# Autodesk Inventor assembly: 3 in 30A flex wheel 36t gear HS mount
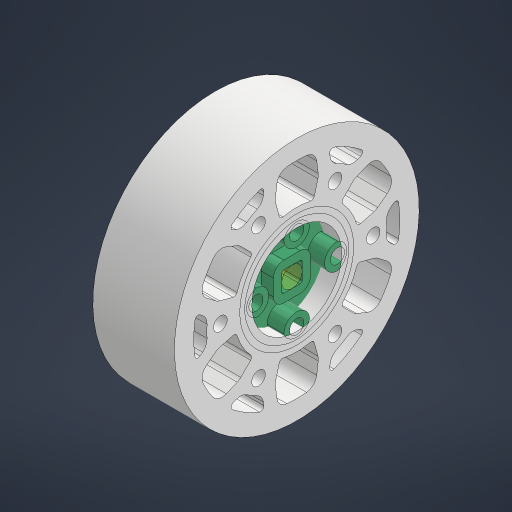
[picture p0: Inventor's stored thumbnail of the model, 512x512]
Saved by Autodesk Inventor 2023.2 (Build 272271030, 271C)
## iProperties
Created: 2023-05-28
Part Number: 3 in 30A flex wheel 36t gear HS mount
Document SubType Name: Assembly
Designer: Main Account
Author: Main Account
## Documents named in this file (4)
- C:\Users\Main Account\InventorProjects\VEX\Custom Library\3 in 30A flex wheel 36t gear HS mount.iam
- C:\Users\Main Account\InventorProjects\VEX\Library Backup\Library 1.4\Motion\Gears\HS Gear\Old Gears\HS 36T Gear, No Insert.ipt
- C:\Users\Main Account\InventorProjects\VEX\Library Backup\Library 1.4\Motion\Wheels\Flex Wheels\3.000 Flex Wheel\3.000 30A 1.000.ipt
- C:\Users\Main Account\InventorProjects\VEX\Library Backup\Library 1.4\Motion\Wheels\Flex Wheels\3.000 Flex Wheel.ipt
## Components (3 placed, 2 different names)
1. HS 36T Gear, No Insert:1 — Mate:1, Mate:2, Rotation:1
2. HS 36T Gear, No Insert:2 — Mate:1, Mate:2, Rotation:1, Mate:3, Flush:1
3. 3.000 30A 1.000:1 — Mate:3, Flush:1
## Relationships (5: Mate 3, RelateRotation 1, Flush 1)
- Mate:1 (-0.0508 mm): HS 36T Gear, No Insert:1 ↔ HS 36T Gear, No Insert:2
- Mate:2: HS 36T Gear, No Insert:1 ↔ HS 36T Gear, No Insert:2
- Rotation:1 [RelateRotation] (1 ul): HS 36T Gear, No Insert:1 ↔ HS 36T Gear, No Insert:2
- Mate:3: HS 36T Gear, No Insert:2 ↔ 3.000 30A 1.000:1
- Flush:1 (-0.0254 mm): HS 36T Gear, No Insert:2 ↔ 3.000 30A 1.000:1
